# Autodesk Inventor assembly: ASY LASEDR NDM VOS
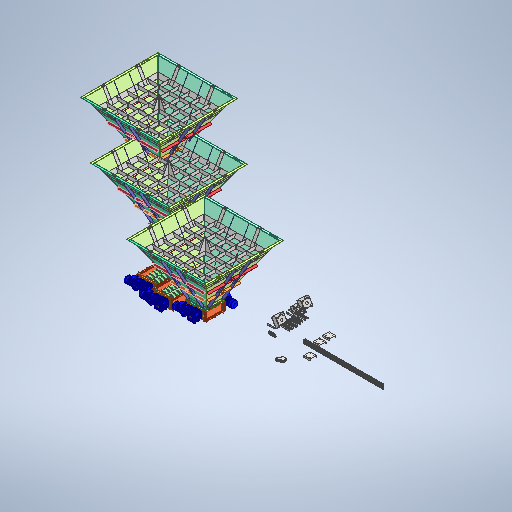
[picture p0: Inventor's stored thumbnail of the model, 512x512]
Saved by Autodesk Inventor 2025 (Build 290162010, 162A)
## iProperties
Created: 2025-01-17
Part Number: ASY LASEDR NDM VOS
Document SubType Name: Assembly
Designer: user
Author: user
## Documents named in this file (11)
- C:\Users\DELL\YandexDisk-badmisterfox\домашниий пк\Inventor\NDM-VOS_powder_hopper\LASER\ASY LASEDR NDM VOS.iam
- C:\Users\DELL\YandexDisk-badmisterfox\домашниий пк\Inventor\NDM-VOS_powder_hopper\Workspaces\Workspace\Cone\ASY MSC 100 cone.iam
- C:\Users\DELL\YandexDisk-badmisterfox\домашниий пк\Inventor\NDM-VOS_powder_hopper\ASY NVPH-400 shredder.iam
- C:\Users\DELL\YandexDisk-badmisterfox\домашниий пк\Inventor\NDM-VOS_powder_hopper\NDM-VOS 777 sredder wall 7.ipt
- C:\Users\DELL\YandexDisk-badmisterfox\домашниий пк\Inventor\NDM-VOS_powder_hopper\NDM-VOS 778 engine plate.ipt
- C:\Users\DELL\YandexDisk-badmisterfox\домашниий пк\Inventor\NDM-VOS_powder_hopper\NDM-VOS 712 flange.ipt
- C:\Users\DELL\YandexDisk-badmisterfox\домашниий пк\Inventor\NDM-VOS_powder_hopper\NDM-VOS 715 flange.ipt
- C:\Users\DELL\YandexDisk-badmisterfox\домашниий пк\Inventor\NDM-VOS_powder_hopper\FL3.6.2  Motor pillar.ipt
- C:\Users\DELL\YandexDisk-badmisterfox\домашниий пк\Inventor\NDM-VOS_powder_hopper\NDM-VOS 913 flange bolt.ipt
- C:\Users\DELL\YandexDisk-badmisterfox\домашниий пк\Inventor\NDM-VOS_powder_hopper\NDM-VOS 912 flange slipway.ipt
- C:\Users\DELL\YandexDisk-badmisterfox\домашниий пк\Inventor\NDM-VOS_powder_hopper\NDM-VOS 901 base plate.ipt
## Components (191 placed, 10 different names)
1. ASY MSC 100 cone.iam:1 [sub-assembly]
2. ASY NVPH-400 shredder.iam:1 [sub-assembly]
3. NDM-VOS 777 sredder wall 7.ipt:1
4. NDM-VOS 778 engine plate.ipt:1
5. NDM-VOS 712 flange.ipt:1
6. NDM-VOS 715 flange.ipt:1
7. FL3.6.2  Motor pillar.ipt:1
8. ASY MSC 100 cone.iam:2 [sub-assembly]
9. ASY MSC 100 cone.iam:3 [sub-assembly]
10. ASY NVPH-400 shredder.iam:2 [sub-assembly]
11. ASY NVPH-400 shredder.iam:3 [sub-assembly]
12. NDM-VOS 777 sredder wall 7.ipt:2
13. NDM-VOS 778 engine plate.ipt:2
14. NDM-VOS 777 sredder wall 7.ipt:3
15. NDM-VOS 778 engine plate.ipt:3
16. NDM-VOS 712 flange.ipt:2
17. NDM-VOS 712 flange.ipt:3
18. NDM-VOS 712 flange.ipt:4
19. NDM-VOS 712 flange.ipt:5
20. NDM-VOS 712 flange.ipt:6
21. NDM-VOS 715 flange.ipt:2
22. NDM-VOS 715 flange.ipt:3
23. NDM-VOS 715 flange.ipt:4
24. NDM-VOS 715 flange.ipt:5
25. NDM-VOS 715 flange.ipt:6
26. FL3.6.2  Motor pillar.ipt:2
27. FL3.6.2  Motor pillar.ipt:3
28. NDM-VOS 901 base plate.ipt:1
29. NDM-VOS 901 base plate.ipt:2
30. NDM-VOS 901 base plate.ipt:3
31. NDM-VOS 901 base plate.ipt:4
32. NDM-VOS 901 base plate.ipt:5
33. NDM-VOS 901 base plate.ipt:6
34. NDM-VOS 901 base plate.ipt:7
35. NDM-VOS 901 base plate.ipt:8
36. NDM-VOS 901 base plate.ipt:9
37. NDM-VOS 901 base plate.ipt:10
38. NDM-VOS 901 base plate.ipt:11
39. NDM-VOS 901 base plate.ipt:12
40. NDM-VOS 912 flange slipway.ipt:1
41. NDM-VOS 912 flange slipway.ipt:2
42. NDM-VOS 912 flange slipway.ipt:3
43. NDM-VOS 912 flange slipway.ipt:4
44. NDM-VOS 912 flange slipway.ipt:5
45. NDM-VOS 912 flange slipway.ipt:6
46. NDM-VOS 912 flange slipway.ipt:7
47. NDM-VOS 912 flange slipway.ipt:8
48. NDM-VOS 912 flange slipway.ipt:9
49. NDM-VOS 912 flange slipway.ipt:10
50. NDM-VOS 912 flange slipway.ipt:11
51. NDM-VOS 912 flange slipway.ipt:12
52. NDM-VOS 912 flange slipway.ipt:13
53. NDM-VOS 912 flange slipway.ipt:14
54. NDM-VOS 912 flange slipway.ipt:15
55. NDM-VOS 912 flange slipway.ipt:16
56. NDM-VOS 912 flange slipway.ipt:17
57. NDM-VOS 912 flange slipway.ipt:18
58. NDM-VOS 912 flange slipway.ipt:19
59. NDM-VOS 912 flange slipway.ipt:20
60. NDM-VOS 912 flange slipway.ipt:21
61. NDM-VOS 912 flange slipway.ipt:22
62. NDM-VOS 912 flange slipway.ipt:23
63. NDM-VOS 912 flange slipway.ipt:24
64. NDM-VOS 912 flange slipway.ipt:25
65. NDM-VOS 912 flange slipway.ipt:26
66. NDM-VOS 912 flange slipway.ipt:27
67. NDM-VOS 912 flange slipway.ipt:28
68. NDM-VOS 912 flange slipway.ipt:29
69. NDM-VOS 912 flange slipway.ipt:30
70. NDM-VOS 912 flange slipway.ipt:31
71. NDM-VOS 912 flange slipway.ipt:32
72. NDM-VOS 912 flange slipway.ipt:33
73. NDM-VOS 912 flange slipway.ipt:34
74. NDM-VOS 912 flange slipway.ipt:35
75. NDM-VOS 912 flange slipway.ipt:36
76. NDM-VOS 912 flange slipway.ipt:37
77. NDM-VOS 912 flange slipway.ipt:38
78. NDM-VOS 912 flange slipway.ipt:39
79. NDM-VOS 912 flange slipway.ipt:40
80. NDM-VOS 912 flange slipway.ipt:41
81. NDM-VOS 912 flange slipway.ipt:42
82. NDM-VOS 912 flange slipway.ipt:43
83. NDM-VOS 912 flange slipway.ipt:44
84. NDM-VOS 912 flange slipway.ipt:45
85. NDM-VOS 912 flange slipway.ipt:46
86. NDM-VOS 912 flange slipway.ipt:47
87. NDM-VOS 912 flange slipway.ipt:48
88. NDM-VOS 912 flange slipway.ipt:49
89. NDM-VOS 912 flange slipway.ipt:50
90. NDM-VOS 912 flange slipway.ipt:51
91. NDM-VOS 912 flange slipway.ipt:52
92. NDM-VOS 912 flange slipway.ipt:53
93. NDM-VOS 912 flange slipway.ipt:54
94. NDM-VOS 912 flange slipway.ipt:55
95. NDM-VOS 912 flange slipway.ipt:56
96. NDM-VOS 912 flange slipway.ipt:57
97. NDM-VOS 912 flange slipway.ipt:58
98. NDM-VOS 912 flange slipway.ipt:59
99. NDM-VOS 912 flange slipway.ipt:60
100. NDM-VOS 912 flange slipway.ipt:61
101. NDM-VOS 912 flange slipway.ipt:62
102. NDM-VOS 912 flange slipway.ipt:63
103. NDM-VOS 912 flange slipway.ipt:64
104. NDM-VOS 912 flange slipway.ipt:65
105. NDM-VOS 912 flange slipway.ipt:66
106. NDM-VOS 912 flange slipway.ipt:67
107. NDM-VOS 912 flange slipway.ipt:68
108. NDM-VOS 912 flange slipway.ipt:69
109. NDM-VOS 912 flange slipway.ipt:70
110. NDM-VOS 912 flange slipway.ipt:71
111. NDM-VOS 912 flange slipway.ipt:72
112. NDM-VOS 912 flange slipway.ipt:73
113. NDM-VOS 912 flange slipway.ipt:74
114. NDM-VOS 912 flange slipway.ipt:75
115. NDM-VOS 912 flange slipway.ipt:76
116. NDM-VOS 912 flange slipway.ipt:77
117. NDM-VOS 912 flange slipway.ipt:78
118. NDM-VOS 912 flange slipway.ipt:79
119. NDM-VOS 912 flange slipway.ipt:80
120. NDM-VOS 912 flange slipway.ipt:81
121. NDM-VOS 912 flange slipway.ipt:82
122. NDM-VOS 912 flange slipway.ipt:83
123. NDM-VOS 912 flange slipway.ipt:84
124. NDM-VOS 912 flange slipway.ipt:85
125. NDM-VOS 912 flange slipway.ipt:86
126. NDM-VOS 912 flange slipway.ipt:87
127. NDM-VOS 912 flange slipway.ipt:88
128. NDM-VOS 912 flange slipway.ipt:89
129. NDM-VOS 912 flange slipway.ipt:90
130. NDM-VOS 912 flange slipway.ipt:91
131. NDM-VOS 912 flange slipway.ipt:92
132. NDM-VOS 913 flange bolt.ipt:1
133. NDM-VOS 913 flange bolt.ipt:2
134. NDM-VOS 913 flange bolt.ipt:3
135. NDM-VOS 913 flange bolt.ipt:4
136. NDM-VOS 913 flange bolt.ipt:5
137. NDM-VOS 913 flange bolt.ipt:6
138. NDM-VOS 913 flange bolt.ipt:7
139. NDM-VOS 913 flange bolt.ipt:8
140. NDM-VOS 913 flange bolt.ipt:9
141. NDM-VOS 913 flange bolt.ipt:10
142. NDM-VOS 913 flange bolt.ipt:11
143. NDM-VOS 913 flange bolt.ipt:12
144. NDM-VOS 913 flange bolt.ipt:13
145. NDM-VOS 913 flange bolt.ipt:14
146. NDM-VOS 913 flange bolt.ipt:15
147. NDM-VOS 913 flange bolt.ipt:16
148. NDM-VOS 913 flange bolt.ipt:17
149. NDM-VOS 913 flange bolt.ipt:18
150. NDM-VOS 913 flange bolt.ipt:19
151. NDM-VOS 913 flange bolt.ipt:20
152. NDM-VOS 913 flange bolt.ipt:21
153. NDM-VOS 913 flange bolt.ipt:22
154. NDM-VOS 913 flange bolt.ipt:23
155. NDM-VOS 913 flange bolt.ipt:24
156. NDM-VOS 913 flange bolt.ipt:25
157. NDM-VOS 913 flange bolt.ipt:26
158. NDM-VOS 913 flange bolt.ipt:27
159. NDM-VOS 913 flange bolt.ipt:28
160. NDM-VOS 913 flange bolt.ipt:29
161. NDM-VOS 913 flange bolt.ipt:30
162. NDM-VOS 913 flange bolt.ipt:31
163. NDM-VOS 913 flange bolt.ipt:32
164. NDM-VOS 913 flange bolt.ipt:33
165. NDM-VOS 913 flange bolt.ipt:34
166. NDM-VOS 913 flange bolt.ipt:35
167. NDM-VOS 913 flange bolt.ipt:36
168. NDM-VOS 913 flange bolt.ipt:37
169. NDM-VOS 913 flange bolt.ipt:38
170. NDM-VOS 913 flange bolt.ipt:39
171. NDM-VOS 913 flange bolt.ipt:40
172. NDM-VOS 913 flange bolt.ipt:41
173. NDM-VOS 913 flange bolt.ipt:42
174. NDM-VOS 913 flange bolt.ipt:43
175. NDM-VOS 913 flange bolt.ipt:44
176. NDM-VOS 913 flange bolt.ipt:45
177. NDM-VOS 913 flange bolt.ipt:46
178. NDM-VOS 913 flange bolt.ipt:47
179. NDM-VOS 913 flange bolt.ipt:48
180. NDM-VOS 913 flange bolt.ipt:49
181. NDM-VOS 913 flange bolt.ipt:50
182. NDM-VOS 913 flange bolt.ipt:51
183. NDM-VOS 913 flange bolt.ipt:52
184. NDM-VOS 913 flange bolt.ipt:53
185. NDM-VOS 913 flange bolt.ipt:54
186. NDM-VOS 913 flange bolt.ipt:55
187. NDM-VOS 913 flange bolt.ipt:56
188. NDM-VOS 913 flange bolt.ipt:57
189. NDM-VOS 913 flange bolt.ipt:58
190. NDM-VOS 913 flange bolt.ipt:59
191. NDM-VOS 913 flange bolt.ipt:60
## Component patterns: (12 elements, first: NDM-VOS 901 base plate.ipt:1), (92 elements, first: NDM-VOS 912 flange slipway.ipt:1), (60 elements, first: NDM-VOS 913 flange bolt.ipt:1)
## Relationships (5: WeldJoint 4, Mate 1)
- [WeldJoint]: ASY MSC 100 cone.iam:1 ↔ ASY NVPH-400 shredder.iam:1
- [WeldJoint]: NDM-VOS 777 sredder wall 7.ipt:1 ↔ NDM-VOS 778 engine plate.ipt:1
- [Mate]: NDM-VOS 778 engine plate.ipt:1 ↔ NDM-VOS 712 flange.ipt:1
- [WeldJoint]: NDM-VOS 777 sredder wall 7.ipt:2 ↔ NDM-VOS 778 engine plate.ipt:2
- [WeldJoint]: NDM-VOS 777 sredder wall 7.ipt:3 ↔ NDM-VOS 778 engine plate.ipt:3
## Named parameters: d3_d209 = 0 mm, d4_d209 = 0 mm
